# Autodesk Inventor assembly: Flywheel Gearbox
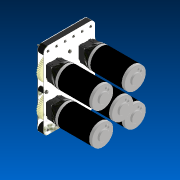
[picture p0: Inventor's stored thumbnail of the model, 180x180]
Saved by Autodesk Inventor 2022 (Build 260153000, 153)
## iProperties
Created: 2022-02-21
Part Number: Flywheel Gearbox
Document SubType Name: Assembly
Designer: omard
Mass: 7293.51 g
Surface Area: 6342.65 cm^2
Volume: 2548.68 cm^3
Density: 2.86168 g/cm^3
Author: omard
## Documents named in this file (21)
- C:\Users\score_nygvs6w\OneDrive - Auburn University\BasketBall Shooting Robot\Flywheel Gearbox.iam
- C:\Users\score_nygvs6w\OneDrive - Auburn University\BasketBall Shooting Robot\VEX Parts\CIM Motor (217-2000).ipt
- C:\Users\score_nygvs6w\OneDrive - Auburn University\BasketBall Shooting Robot\VEX Parts\VersaPlanetary v2 NoStage.iam
- C:\Users\score_nygvs6w\OneDrive - Auburn University\BasketBall Shooting Robot\VEX Parts\54T Aluminum Spur Gear (20 DP, 1_2 Hex Bore) (217-3573).ipt
- C:\Users\score_nygvs6w\OneDrive - Auburn University\BasketBall Shooting Robot\VEX Parts\54T Aluminum Spur Gear (20 DP, 1_2 Hex Bore, VersaKeys) (217-3221).ipt
- C:\Users\score_nygvs6w\OneDrive - Auburn University\BasketBall Shooting Robot\VEX Parts\Clamping Shaft Collar - 1_2 Hex ID (217-2737).ipt
- C:\Users\score_nygvs6w\OneDrive - Auburn University\BasketBall Shooting Robot\VEX Parts\60T x 18mm Wide VersaPulley Kit (HTD 5mm, VersaKeys) (217-3200).iam
- C:\Users\score_nygvs6w\OneDrive - Auburn University\BasketBall Shooting Robot\VEX Parts\1_2” Hex Bore Aluminum VersaHub (217-2592).ipt
- C:\Users\score_nygvs6w\OneDrive - Auburn University\BasketBall Shooting Robot\VEX Parts\1.125 Bearing Pilot Plastic VersaHub (1_4 Wide, w_ Plate Sprocket Mount) (217-3234).ipt
- C:\Users\score_nygvs6w\OneDrive - Auburn University\BasketBall Shooting Robot\Motor Bracket Outer Panel.ipt
- C:\Users\score_nygvs6w\OneDrive - Auburn University\BasketBall Shooting Robot\Motor Bracket Inner Panel.ipt
- C:\Users\score_nygvs6w\OneDrive - Auburn University\BasketBall Shooting Robot\VEX Parts\#8-32 x 0.625 Star Drive Screw (276-4993).ipt
- C:\Users\score_nygvs6w\OneDrive - Auburn University\BasketBall Shooting Robot\Motor Bracket Seperator.ipt
- C:\Users\score_nygvs6w\OneDrive - Auburn University\BasketBall Shooting Robot\VEX Parts\13.75mm (1_2 ThunderHex ID) x 1.125 OD x 0.313 WD (Flanged Bearing) (217-4006).ipt
- C:\Users\score_nygvs6w\OneDrive - Auburn University\BasketBall Shooting Robot\1_10 Spacer 1_2 Hex Custom.ipt
- C:\Users\score_nygvs6w\OneDrive - Auburn University\BasketBall Shooting Robot\VEX Parts\#8-32 x 1.250 Star Drive Screw (276-4997).ipt
- C:\Users\score_nygvs6w\OneDrive - Auburn University\BasketBall Shooting Robot\VEX Parts\#8-32 Nylock Nut (275-1027).ipt
- C:\Users\score_nygvs6w\OneDrive - Auburn University\BasketBall Shooting Robot\5_8 Spacer Screw Custom.ipt
- C:\Users\score_nygvs6w\OneDrive - Auburn University\BasketBall Shooting Robot\VEX Parts\#8-32 x 1.000 Star Drive Screw (276-4996).ipt
- C:\Users\score_nygvs6w\OneDrive - Auburn University\BasketBall Shooting Robot\VEX Parts\Falcon 500, Powered by Talon FX (217-6515).iam
- C:\Users\score_nygvs6w\OneDrive - Auburn University\BasketBall Shooting Robot\VEX Parts\VersaPlanetary v2 NoStage Encoder.iam
## Components (84 placed, 20 different names)
1. CIM Motor (217-2000):1 — Mate:5, Mate:6, Mate:18, Flush:10
2. CIM Motor (217-2000):2 — Flush:2, Mate:11, Mate:12, Mate:14, Mate:16, Mate:19, Mate:56
3. CIM Motor (217-2000):3 — Mate:7, Mate:8, Mate:15, Mate:18, Mate:19, Mate:54, Mate:55
4. CIM Motor (217-2000):4 — Flush:2, Mate:9, Mate:10, Mate:13, Mate:55, Flush:10, Flush:11
5. CIM Motor (217-2000):5 — Mate:54, Flush:11, Mate:56
6. VersaPlanetary v2 NoStage Encoder:1 [sub-assembly] — Angle:2, Mate:7, Mate:8, Mate:15, Mate:25, Angle:5, Mate:47, Angle:15, Mate:48, Mate:51, Angle:16, Mate:60, Mate:62, Angle:29, Mate:105, Mate:110, Angle:32, Mate:113, Mate:189, Mate:199
7. VersaPlanetary v2 NoStage:2 [sub-assembly] — Angle:3, Angle:4, Mate:11, Mate:12, Mate:14, Mate:23, Angle:7, Angle:10, Mate:59, Mate:99, Angle:30, Mate:106, Mate:112, Mate:187, Mate:193, Mate:200
8. VersaPlanetary v2 NoStage:3 [sub-assembly] — Mate:5, Angle:1, Angle:2, Angle:3, Mate:6, Mate:22, Angle:6, Mate:58, Mate:66, Mate:98, Angle:31, Mate:107, Mate:111, Mate:191, Mate:192, Mate:196, Mate:197, Flush:12
9. VersaPlanetary v2 NoStage:4 [sub-assembly] — Angle:4, Mate:9, Mate:10, Mate:13, Mate:24, Angle:8, Flush:8, Mate:57, Mate:97, Angle:27, Mate:103, Mate:108, Mate:190, Mate:195, Mate:198, Flush:12
10. VersaPlanetary v2 NoStage:5 [sub-assembly] — Flush:8, Angle:10, Mate:61, Mate:100, Angle:28, Mate:104, Mate:109, Mate:188, Mate:194, Mate:201, Mate:202
11. 54T Aluminum Spur Gear (20 DP, 1_2 Hex Bore) (217-3573):1 — Mate:22, Angle:6, Flush:6, Mate:102
12. 54T Aluminum Spur Gear (20 DP, 1_2 Hex Bore, VersaKeys) (217-3221):1 — Mate:25, Angle:5, Flush:4, Mate:49, Mate:50, Mate:52
13. 54T Aluminum Spur Gear (20 DP, 1_2 Hex Bore) (217-3573):2 — Mate:23, Angle:7, Flush:5, Flush:6
14. 54T Aluminum Spur Gear (20 DP, 1_2 Hex Bore) (217-3573):3 — Mate:24, Angle:8, Flush:4, Flush:5, Flush:7
15. 54T Aluminum Spur Gear (20 DP, 1_2 Hex Bore) (217-3573):4 — Flush:7
16. Clamping Shaft Collar - 1_2 Hex ID (217-2737):5 — Mate:51, Angle:16, Mate:52
17. 60T x 18mm Wide VersaPulley Kit (HTD 5mm, VersaKeys) (217-3200):1 [sub-assembly] — Mate:41, Mate:42, Mate:46, Mate:53, Mate:133, Mate:134, Mate:135, Mate:136, Mate:137, Mate:138, Angle:39, Angle:40, Angle:41, Angle:42, Angle:43, Angle:44
18. 1_2” Hex Bore Aluminum VersaHub (217-2592):1 — Mate:41, Mate:42, Mate:46, Mate:47, Angle:15, Mate:114, Mate:115, Mate:116, Mate:117, Mate:118, Mate:119, Mate:120, Mate:121, Mate:122, Mate:123, Mate:124, Mate:125, Mate:126
19. 1.125 Bearing Pilot Plastic VersaHub (1_4 Wide, w_ Plate Sprocket Mount) (217-3234):1 — Mate:48, Mate:49, Mate:50, Mate:53
20. Motor Bracket Outer Panel:1 — Mate:89, Mate:90, Mate:91, Mate:92, Mate:93, Mate:94, Mate:95, Mate:96, Mate:101, Mate:171, Mate:172, Mate:173, Mate:174, Mate:175, Mate:176, Mate:177, Mate:178, Angle:65, Angle:66, Angle:67, Angle:68
21. Motor Bracket Inner Panel:1 — Mate:57, Mate:58, Mate:59, Mate:60, Mate:61, Mate:62, Mate:63, Mate:64, Mate:65, Mate:67, Mate:68, Mate:69, Mate:70, Mate:71, Mate:72, Mate:73, Mate:74, Mate:75, Mate:76, Mate:77, Mate:78, Mate:79, Mate:80, Mate:81, Mate:82, Angle:17, Angle:18, Angle:19, Angle:20, Angle:21, Angle:22, Angle:23, Angle:24, Angle:25, Angle:26, Mate:83, Mate:84, Mate:85, Mate:86, Mate:87, Mate:88, Angle:33, Angle:34, Angle:35, Angle:36, Angle:37, Angle:38, Angle:45, Angle:46, Angle:47, Angle:48, Mate:139, Mate:140, Mate:141, Mate:142, Mate:143, Mate:144, Mate:145, Mate:146, Mate:147, Mate:148, Mate:149, Mate:150, Mate:151, Mate:152, Mate:153, Mate:154, Mate:155, Mate:156, Mate:157, Mate:158, Mate:159, Mate:160, Mate:161, Mate:162, Angle:49, Angle:50, Angle:51, Angle:52, Angle:53, Angle:54, Angle:55, Angle:56, Angle:57, Angle:58, Angle:59, Angle:60, Mate:163, Mate:164, Mate:165, Mate:166, Mate:167, Mate:168, Mate:169, Mate:170, Angle:61, Angle:62, Angle:63, Angle:64, Mate:183, Mate:184, Mate:185, Mate:186, Angle:69, Angle:70, Angle:71, Angle:72, Mate:202
22. #8-32 x 0.625 Star Drive Screw (276-4993):1 — Mate:65, Mate:81, Angle:26
23. #8-32 x 0.625 Star Drive Screw (276-4993):2 — Mate:66, Mate:82, Angle:25
24. #8-32 x 0.625 Star Drive Screw (276-4993):3 — Mate:63, Mate:80, Angle:24
25. #8-32 x 0.625 Star Drive Screw (276-4993):4 — Mate:64, Mate:79, Angle:23
26. #8-32 x 0.625 Star Drive Screw (276-4993):5 — Mate:72, Mate:73, Angle:22
27. #8-32 x 0.625 Star Drive Screw (276-4993):6 — Mate:71, Mate:74, Angle:21
28. #8-32 x 0.625 Star Drive Screw (276-4993):7 — Mate:68, Mate:76, Angle:20
29. #8-32 x 0.625 Star Drive Screw (276-4993):8 — Mate:67, Mate:75, Angle:19
30. #8-32 x 0.625 Star Drive Screw (276-4993):9 — Mate:70, Mate:78, Angle:18
31. #8-32 x 0.625 Star Drive Screw (276-4993):10 — Mate:69, Mate:77, Angle:17
32. Motor Bracket Seperator:1 — Mate:83, Mate:84, Mate:88
33. Motor Bracket Seperator:2 — Mate:85, Mate:86, Mate:87, Mate:101
34. 13.75mm (1_2 ThunderHex ID) x 1.125 OD x 0.313 WD (Flanged Bearing) (217-4006):1 — Mate:89, Mate:94, Mate:98, Mate:102, Angle:48
35. 13.75mm (1_2 ThunderHex ID) x 1.125 OD x 0.313 WD (Flanged Bearing) (217-4006):2 — Mate:90, Mate:95, Mate:97, Angle:47
36. 13.75mm (1_2 ThunderHex ID) x 1.125 OD x 0.313 WD (Flanged Bearing) (217-4006):3 — Mate:92, Mate:96, Mate:100, Angle:46
37. 13.75mm (1_2 ThunderHex ID) x 1.125 OD x 0.313 WD (Flanged Bearing) (217-4006):4 — Mate:91, Mate:93, Mate:99, Angle:45
38. 1_10 Spacer 1_2 Hex Custom:1 — Angle:27, Mate:104, Mate:109
39. 1_10 Spacer 1_2 Hex Custom:2 — Angle:30, Mate:106, Mate:112
40. 1_10 Spacer 1_2 Hex Custom:3 — Angle:31, Mate:107, Mate:111
41. 1_10 Spacer 1_2 Hex Custom:4 — Angle:29, Mate:105, Mate:110
42. 1_10 Spacer 1_2 Hex Custom:5 — Angle:28, Mate:103, Mate:108
43. 1_10 Spacer 1_2 Hex Custom:6 — Angle:32, Mate:113, Mate:114
44. #8-32 x 1.250 Star Drive Screw (276-4997):1 — Mate:120, Mate:124, Angle:38, Mate:127
45. #8-32 x 1.250 Star Drive Screw (276-4997):2 — Mate:116, Mate:123, Angle:37, Mate:128
46. #8-32 x 1.250 Star Drive Screw (276-4997):3 — Mate:118, Mate:125, Angle:36, Mate:130
47. #8-32 x 1.250 Star Drive Screw (276-4997):4 — Mate:115, Mate:121, Angle:35, Mate:131
48. #8-32 x 1.250 Star Drive Screw (276-4997):5 — Mate:117, Mate:122, Angle:34, Mate:132
49. #8-32 x 1.250 Star Drive Screw (276-4997):6 — Mate:119, Mate:126, Angle:33, Mate:129
50. #8-32 Nylock Nut (275-1027):1 — Mate:128, Mate:134, Angle:43
51. #8-32 Nylock Nut (275-1027):2 — Mate:129, Mate:136, Angle:42
52. #8-32 Nylock Nut (275-1027):3 — Mate:132, Mate:138, Angle:39
53. #8-32 Nylock Nut (275-1027):4 — Mate:131, Mate:133, Angle:40
54. #8-32 Nylock Nut (275-1027):5 — Mate:130, Mate:137, Angle:41
55. #8-32 Nylock Nut (275-1027):6 — Mate:127, Mate:135, Angle:44
56. #8-32 x 1.250 Star Drive Screw (276-4997):7 — Mate:144, Mate:162, Angle:60
57. #8-32 x 1.250 Star Drive Screw (276-4997):8 — Mate:143, Mate:161, Angle:58
58. #8-32 x 1.250 Star Drive Screw (276-4997):9 — Mate:141, Mate:159, Angle:59
59. #8-32 x 1.250 Star Drive Screw (276-4997):10 — Mate:140, Mate:158, Angle:57
60. #8-32 x 1.250 Star Drive Screw (276-4997):11 — Mate:142, Mate:160, Angle:56
61. #8-32 x 1.250 Star Drive Screw (276-4997):12 — Mate:139, Mate:157, Angle:55
62. #8-32 x 1.250 Star Drive Screw (276-4997):13 — Mate:145, Mate:151, Angle:54
63. #8-32 x 1.250 Star Drive Screw (276-4997):14 — Mate:146, Mate:152, Angle:53
64. #8-32 x 1.250 Star Drive Screw (276-4997):15 — Mate:147, Mate:153, Angle:52
65. #8-32 x 1.250 Star Drive Screw (276-4997):16 — Mate:148, Mate:154, Angle:51
66. #8-32 x 1.250 Star Drive Screw (276-4997):17 — Mate:149, Mate:155, Angle:50
67. #8-32 x 1.250 Star Drive Screw (276-4997):18 — Mate:150, Mate:156, Angle:49
68. 5_8 Spacer Screw Custom:1 — Mate:165, Mate:168, Angle:64
69. 5_8 Spacer Screw Custom:2 — Mate:166, Mate:167, Angle:63
70. 5_8 Spacer Screw Custom:3 — Mate:164, Mate:169, Angle:62
71. 5_8 Spacer Screw Custom:4 — Mate:163, Mate:170, Angle:61
72. #8-32 x 1.000 Star Drive Screw (276-4996):1 — Mate:171, Mate:172, Angle:65, Mate:181
73. #8-32 x 1.000 Star Drive Screw (276-4996):2 — Mate:173, Mate:174, Angle:66, Mate:179
74. #8-32 x 1.000 Star Drive Screw (276-4996):3 — Mate:177, Mate:178, Angle:68, Mate:182
75. #8-32 x 1.000 Star Drive Screw (276-4996):4 — Mate:175, Mate:176, Angle:67, Mate:180
76. #8-32 Nylock Nut (275-1027):7 — Mate:179, Mate:184, Angle:71
77. #8-32 Nylock Nut (275-1027):8 — Mate:180, Mate:183, Angle:72
78. #8-32 Nylock Nut (275-1027):9 — Mate:181, Mate:185, Angle:70
79. #8-32 Nylock Nut (275-1027):10 — Mate:182, Mate:186, Angle:69
80. Falcon 500, Powered by Talon FX (217-6515):1 [sub-assembly] — Mate:187, Mate:193, Mate:200
81. Falcon 500, Powered by Talon FX (217-6515):2 [sub-assembly] — Mate:189, Mate:199
82. Falcon 500, Powered by Talon FX (217-6515):3 [sub-assembly] — Mate:190, Mate:195, Mate:198
83. Falcon 500, Powered by Talon FX (217-6515):4 [sub-assembly] — Mate:191, Mate:192, Mate:196, Mate:197
84. Falcon 500, Powered by Talon FX (217-6515):5 [sub-assembly] — Mate:188, Mate:194, Mate:201
## Relationships (258: Mate 181, Angle 68, Flush 9)
- Flush:2: CIM Motor (217-2000):2 ↔ CIM Motor (217-2000):4
- Mate:5: CIM Motor (217-2000):1 ↔ VersaPlanetary v2 NoStage:3
- Angle:1 (0 deg): VersaPlanetary v2 NoStage:3
- Angle:2 (0 deg): VersaPlanetary v2 NoStage Encoder:1 ↔ VersaPlanetary v2 NoStage:3
- Angle:3 (0 deg): VersaPlanetary v2 NoStage:2 ↔ VersaPlanetary v2 NoStage:3
- Angle:4 (0 deg): VersaPlanetary v2 NoStage:2 ↔ VersaPlanetary v2 NoStage:4
- Mate:6: CIM Motor (217-2000):1 ↔ VersaPlanetary v2 NoStage:3
- Mate:7: CIM Motor (217-2000):3 ↔ VersaPlanetary v2 NoStage Encoder:1
- Mate:8: CIM Motor (217-2000):3 ↔ VersaPlanetary v2 NoStage Encoder:1
- Mate:9: CIM Motor (217-2000):4 ↔ VersaPlanetary v2 NoStage:4
- Mate:10: CIM Motor (217-2000):4 ↔ VersaPlanetary v2 NoStage:4
- Mate:11: CIM Motor (217-2000):2 ↔ VersaPlanetary v2 NoStage:2
- Mate:12: CIM Motor (217-2000):2 ↔ VersaPlanetary v2 NoStage:2
- Mate:13: CIM Motor (217-2000):4 ↔ VersaPlanetary v2 NoStage:4
- Mate:14: CIM Motor (217-2000):2 ↔ VersaPlanetary v2 NoStage:2
- Mate:15: CIM Motor (217-2000):3 ↔ VersaPlanetary v2 NoStage Encoder:1
- Mate:16: CIM Motor (217-2000):2
- Mate:18 (68.58 mm): CIM Motor (217-2000):1 ↔ CIM Motor (217-2000):3
- Mate:19 (68.58 mm): CIM Motor (217-2000):2 ↔ CIM Motor (217-2000):3
- Mate:22: VersaPlanetary v2 NoStage:3 ↔ 54T Aluminum Spur Gear (20 DP, 1_2 Hex Bore) (217-3573):1
- Mate:23: VersaPlanetary v2 NoStage:2 ↔ 54T Aluminum Spur Gear (20 DP, 1_2 Hex Bore) (217-3573):2
- Mate:24: VersaPlanetary v2 NoStage:4 ↔ 54T Aluminum Spur Gear (20 DP, 1_2 Hex Bore) (217-3573):3
- Mate:25: VersaPlanetary v2 NoStage Encoder:1 ↔ 54T Aluminum Spur Gear (20 DP, 1_2 Hex Bore, VersaKeys) (217-3221):1
- Angle:5 (0 deg): VersaPlanetary v2 NoStage Encoder:1 ↔ 54T Aluminum Spur Gear (20 DP, 1_2 Hex Bore, VersaKeys) (217-3221):1
- Angle:6 (0 deg): VersaPlanetary v2 NoStage:3 ↔ 54T Aluminum Spur Gear (20 DP, 1_2 Hex Bore) (217-3573):1
- Angle:7 (0 deg): VersaPlanetary v2 NoStage:2 ↔ 54T Aluminum Spur Gear (20 DP, 1_2 Hex Bore) (217-3573):2
- Angle:8 (0 deg): VersaPlanetary v2 NoStage:4 ↔ 54T Aluminum Spur Gear (20 DP, 1_2 Hex Bore) (217-3573):3
- Flush:4: 54T Aluminum Spur Gear (20 DP, 1_2 Hex Bore, VersaKeys) (217-3221):1 ↔ 54T Aluminum Spur Gear (20 DP, 1_2 Hex Bore) (217-3573):3
- Flush:5: 54T Aluminum Spur Gear (20 DP, 1_2 Hex Bore) (217-3573):2 ↔ 54T Aluminum Spur Gear (20 DP, 1_2 Hex Bore) (217-3573):3
- Flush:6: 54T Aluminum Spur Gear (20 DP, 1_2 Hex Bore) (217-3573):1 ↔ 54T Aluminum Spur Gear (20 DP, 1_2 Hex Bore) (217-3573):2
- [Mate]: CIM Motor (217-2000):5 ↔ VersaPlanetary v2 NoStage:5
- [Mate]: CIM Motor (217-2000):5 ↔ VersaPlanetary v2 NoStage:5
- [Mate]: CIM Motor (217-2000):5 ↔ VersaPlanetary v2 NoStage:5
- [Mate]: VersaPlanetary v2 NoStage:5 ↔ 54T Aluminum Spur Gear (20 DP, 1_2 Hex Bore) (217-3573):4
- [Angle] (0 deg): VersaPlanetary v2 NoStage:5 ↔ 54T Aluminum Spur Gear (20 DP, 1_2 Hex Bore) (217-3573):4
- Flush:7: 54T Aluminum Spur Gear (20 DP, 1_2 Hex Bore) (217-3573):3 ↔ 54T Aluminum Spur Gear (20 DP, 1_2 Hex Bore) (217-3573):4
- Flush:8: VersaPlanetary v2 NoStage:4 ↔ VersaPlanetary v2 NoStage:5
- Angle:10 (0 deg): VersaPlanetary v2 NoStage:2 ↔ VersaPlanetary v2 NoStage:5
- Mate:41: 60T x 18mm Wide VersaPulley Kit (HTD 5mm, VersaKeys) (217-3200):1 ↔ 1_2” Hex Bore Aluminum VersaHub (217-2592):1
- Mate:42: 60T x 18mm Wide VersaPulley Kit (HTD 5mm, VersaKeys) (217-3200):1 ↔ 1_2” Hex Bore Aluminum VersaHub (217-2592):1
- Mate:46: 60T x 18mm Wide VersaPulley Kit (HTD 5mm, VersaKeys) (217-3200):1 ↔ 1_2” Hex Bore Aluminum VersaHub (217-2592):1
- Mate:47: VersaPlanetary v2 NoStage Encoder:1 ↔ 1_2” Hex Bore Aluminum VersaHub (217-2592):1
- Angle:15 (0 deg): VersaPlanetary v2 NoStage Encoder:1 ↔ 1_2” Hex Bore Aluminum VersaHub (217-2592):1
- Mate:48: VersaPlanetary v2 NoStage Encoder:1 ↔ 1.125 Bearing Pilot Plastic VersaHub (1_4 Wide, w_ Plate Sprocket Mount) (217-3234):1
- Mate:49: 54T Aluminum Spur Gear (20 DP, 1_2 Hex Bore, VersaKeys) (217-3221):1 ↔ 1.125 Bearing Pilot Plastic VersaHub (1_4 Wide, w_ Plate Sprocket Mount) (217-3234):1
- Mate:50: 54T Aluminum Spur Gear (20 DP, 1_2 Hex Bore, VersaKeys) (217-3221):1 ↔ 1.125 Bearing Pilot Plastic VersaHub (1_4 Wide, w_ Plate Sprocket Mount) (217-3234):1
- Mate:51: VersaPlanetary v2 NoStage Encoder:1 ↔ Clamping Shaft Collar - 1_2 Hex ID (217-2737):5
- Angle:16 (0 deg): VersaPlanetary v2 NoStage Encoder:1 ↔ Clamping Shaft Collar - 1_2 Hex ID (217-2737):5
- Mate:52: 54T Aluminum Spur Gear (20 DP, 1_2 Hex Bore, VersaKeys) (217-3221):1 ↔ Clamping Shaft Collar - 1_2 Hex ID (217-2737):5
- Mate:53: 60T x 18mm Wide VersaPulley Kit (HTD 5mm, VersaKeys) (217-3200):1 ↔ 1.125 Bearing Pilot Plastic VersaHub (1_4 Wide, w_ Plate Sprocket Mount) (217-3234):1
- Mate:54 (68.58 mm): CIM Motor (217-2000):3 ↔ CIM Motor (217-2000):5
- Mate:55 (68.58 mm): CIM Motor (217-2000):3 ↔ CIM Motor (217-2000):4
- Flush:10: CIM Motor (217-2000):1 ↔ CIM Motor (217-2000):4
- Flush:11: CIM Motor (217-2000):4 ↔ CIM Motor (217-2000):5
- Mate:56 (96.9868 mm): CIM Motor (217-2000):2 ↔ CIM Motor (217-2000):5
- Mate:57: VersaPlanetary v2 NoStage:4 ↔ Motor Bracket Inner Panel:1
- Mate:58: VersaPlanetary v2 NoStage:3 ↔ Motor Bracket Inner Panel:1
- Mate:59: VersaPlanetary v2 NoStage:2 ↔ Motor Bracket Inner Panel:1
- Mate:60: VersaPlanetary v2 NoStage Encoder:1 ↔ Motor Bracket Inner Panel:1
- Mate:61: VersaPlanetary v2 NoStage:5 ↔ Motor Bracket Inner Panel:1
- Mate:62: VersaPlanetary v2 NoStage Encoder:1 ↔ Motor Bracket Inner Panel:1
- Mate:63: Motor Bracket Inner Panel:1 ↔ #8-32 x 0.625 Star Drive Screw (276-4993):3
- Mate:64: Motor Bracket Inner Panel:1 ↔ #8-32 x 0.625 Star Drive Screw (276-4993):4
- Mate:65: Motor Bracket Inner Panel:1 ↔ #8-32 x 0.625 Star Drive Screw (276-4993):1
- Mate:66: VersaPlanetary v2 NoStage:3 ↔ #8-32 x 0.625 Star Drive Screw (276-4993):2
- Mate:67: Motor Bracket Inner Panel:1 ↔ #8-32 x 0.625 Star Drive Screw (276-4993):8
- Mate:68: Motor Bracket Inner Panel:1 ↔ #8-32 x 0.625 Star Drive Screw (276-4993):7
- Mate:69: Motor Bracket Inner Panel:1 ↔ #8-32 x 0.625 Star Drive Screw (276-4993):10
- Mate:70: Motor Bracket Inner Panel:1 ↔ #8-32 x 0.625 Star Drive Screw (276-4993):9
- Mate:71: Motor Bracket Inner Panel:1 ↔ #8-32 x 0.625 Star Drive Screw (276-4993):6
- Mate:72: Motor Bracket Inner Panel:1 ↔ #8-32 x 0.625 Star Drive Screw (276-4993):5
- Mate:73: Motor Bracket Inner Panel:1 ↔ #8-32 x 0.625 Star Drive Screw (276-4993):5
- Mate:74: Motor Bracket Inner Panel:1 ↔ #8-32 x 0.625 Star Drive Screw (276-4993):6
- Mate:75: Motor Bracket Inner Panel:1 ↔ #8-32 x 0.625 Star Drive Screw (276-4993):8
- Mate:76: Motor Bracket Inner Panel:1 ↔ #8-32 x 0.625 Star Drive Screw (276-4993):7
- Mate:77: Motor Bracket Inner Panel:1 ↔ #8-32 x 0.625 Star Drive Screw (276-4993):10
- Mate:78: Motor Bracket Inner Panel:1 ↔ #8-32 x 0.625 Star Drive Screw (276-4993):9
- Mate:79: Motor Bracket Inner Panel:1 ↔ #8-32 x 0.625 Star Drive Screw (276-4993):4
- Mate:80: Motor Bracket Inner Panel:1 ↔ #8-32 x 0.625 Star Drive Screw (276-4993):3
- Mate:81: Motor Bracket Inner Panel:1 ↔ #8-32 x 0.625 Star Drive Screw (276-4993):1
- Mate:82: Motor Bracket Inner Panel:1 ↔ #8-32 x 0.625 Star Drive Screw (276-4993):2
- Angle:17 (0 deg): Motor Bracket Inner Panel:1 ↔ #8-32 x 0.625 Star Drive Screw (276-4993):10
- Angle:18 (0 deg): Motor Bracket Inner Panel:1 ↔ #8-32 x 0.625 Star Drive Screw (276-4993):9
- Angle:19 (0 deg): Motor Bracket Inner Panel:1 ↔ #8-32 x 0.625 Star Drive Screw (276-4993):8
- Angle:20 (0 deg): Motor Bracket Inner Panel:1 ↔ #8-32 x 0.625 Star Drive Screw (276-4993):7
- Angle:21 (0 deg): Motor Bracket Inner Panel:1 ↔ #8-32 x 0.625 Star Drive Screw (276-4993):6
- Angle:22 (0 deg): Motor Bracket Inner Panel:1 ↔ #8-32 x 0.625 Star Drive Screw (276-4993):5
- Angle:23 (0 deg): Motor Bracket Inner Panel:1 ↔ #8-32 x 0.625 Star Drive Screw (276-4993):4
- Angle:24 (0 deg): Motor Bracket Inner Panel:1 ↔ #8-32 x 0.625 Star Drive Screw (276-4993):3
- Angle:25 (0 deg): Motor Bracket Inner Panel:1 ↔ #8-32 x 0.625 Star Drive Screw (276-4993):2
- Angle:26 (0 deg): Motor Bracket Inner Panel:1 ↔ #8-32 x 0.625 Star Drive Screw (276-4993):1
- Mate:83: Motor Bracket Inner Panel:1 ↔ Motor Bracket Seperator:1
- Mate:84: Motor Bracket Inner Panel:1 ↔ Motor Bracket Seperator:1
- Mate:85: Motor Bracket Inner Panel:1 ↔ Motor Bracket Seperator:2
- Mate:86: Motor Bracket Inner Panel:1 ↔ Motor Bracket Seperator:2
- Mate:87: Motor Bracket Inner Panel:1 ↔ Motor Bracket Seperator:2
- Mate:88: Motor Bracket Inner Panel:1 ↔ Motor Bracket Seperator:1
- Mate:89: Motor Bracket Outer Panel:1 ↔ 13.75mm (1_2 ThunderHex ID) x 1.125 OD x 0.313 WD (Flanged Bearing) (217-4006):1
- Mate:90: Motor Bracket Outer Panel:1 ↔ 13.75mm (1_2 ThunderHex ID) x 1.125 OD x 0.313 WD (Flanged Bearing) (217-4006):2
- Mate:91: Motor Bracket Outer Panel:1 ↔ 13.75mm (1_2 ThunderHex ID) x 1.125 OD x 0.313 WD (Flanged Bearing) (217-4006):4
- Mate:92: Motor Bracket Outer Panel:1 ↔ 13.75mm (1_2 ThunderHex ID) x 1.125 OD x 0.313 WD (Flanged Bearing) (217-4006):3
- Mate:93: Motor Bracket Outer Panel:1 ↔ 13.75mm (1_2 ThunderHex ID) x 1.125 OD x 0.313 WD (Flanged Bearing) (217-4006):4
- Mate:94: Motor Bracket Outer Panel:1 ↔ 13.75mm (1_2 ThunderHex ID) x 1.125 OD x 0.313 WD (Flanged Bearing) (217-4006):1
- Mate:95: Motor Bracket Outer Panel:1 ↔ 13.75mm (1_2 ThunderHex ID) x 1.125 OD x 0.313 WD (Flanged Bearing) (217-4006):2
- Mate:96: Motor Bracket Outer Panel:1 ↔ 13.75mm (1_2 ThunderHex ID) x 1.125 OD x 0.313 WD (Flanged Bearing) (217-4006):3
- Mate:97: VersaPlanetary v2 NoStage:4 ↔ 13.75mm (1_2 ThunderHex ID) x 1.125 OD x 0.313 WD (Flanged Bearing) (217-4006):2
- Mate:98: VersaPlanetary v2 NoStage:3 ↔ 13.75mm (1_2 ThunderHex ID) x 1.125 OD x 0.313 WD (Flanged Bearing) (217-4006):1
- Mate:99: VersaPlanetary v2 NoStage:2 ↔ 13.75mm (1_2 ThunderHex ID) x 1.125 OD x 0.313 WD (Flanged Bearing) (217-4006):4
- Mate:100: VersaPlanetary v2 NoStage:5 ↔ 13.75mm (1_2 ThunderHex ID) x 1.125 OD x 0.313 WD (Flanged Bearing) (217-4006):3
- Mate:101: Motor Bracket Outer Panel:1 ↔ Motor Bracket Seperator:2
- Mate:102: 54T Aluminum Spur Gear (20 DP, 1_2 Hex Bore) (217-3573):1 ↔ 13.75mm (1_2 ThunderHex ID) x 1.125 OD x 0.313 WD (Flanged Bearing) (217-4006):1
- Angle:27 (0 deg): VersaPlanetary v2 NoStage:4 ↔ 1_10 Spacer 1_2 Hex Custom:1
- Angle:28 (0 deg): VersaPlanetary v2 NoStage:5 ↔ 1_10 Spacer 1_2 Hex Custom:5
- Angle:29 (0 deg): VersaPlanetary v2 NoStage Encoder:1 ↔ 1_10 Spacer 1_2 Hex Custom:4
- Angle:30 (0 deg): VersaPlanetary v2 NoStage:2 ↔ 1_10 Spacer 1_2 Hex Custom:2
- Angle:31 (0 deg): VersaPlanetary v2 NoStage:3 ↔ 1_10 Spacer 1_2 Hex Custom:3
- Mate:103: VersaPlanetary v2 NoStage:4 ↔ 1_10 Spacer 1_2 Hex Custom:5
- Mate:104: VersaPlanetary v2 NoStage:5 ↔ 1_10 Spacer 1_2 Hex Custom:1
- Mate:105: VersaPlanetary v2 NoStage Encoder:1 ↔ 1_10 Spacer 1_2 Hex Custom:4
- Mate:106: VersaPlanetary v2 NoStage:2 ↔ 1_10 Spacer 1_2 Hex Custom:2
- Mate:107: VersaPlanetary v2 NoStage:3 ↔ 1_10 Spacer 1_2 Hex Custom:3
- Mate:108: VersaPlanetary v2 NoStage:4 ↔ 1_10 Spacer 1_2 Hex Custom:5
- Mate:109: VersaPlanetary v2 NoStage:5 ↔ 1_10 Spacer 1_2 Hex Custom:1
- Mate:110: VersaPlanetary v2 NoStage Encoder:1 ↔ 1_10 Spacer 1_2 Hex Custom:4
- Mate:111: VersaPlanetary v2 NoStage:3 ↔ 1_10 Spacer 1_2 Hex Custom:3
- Mate:112: VersaPlanetary v2 NoStage:2 ↔ 1_10 Spacer 1_2 Hex Custom:2
- Angle:32 (0 deg): VersaPlanetary v2 NoStage Encoder:1 ↔ 1_10 Spacer 1_2 Hex Custom:6
- Mate:113: VersaPlanetary v2 NoStage Encoder:1 ↔ 1_10 Spacer 1_2 Hex Custom:6
- Mate:114: 1_2” Hex Bore Aluminum VersaHub (217-2592):1 ↔ 1_10 Spacer 1_2 Hex Custom:6
- Mate:115: 1_2” Hex Bore Aluminum VersaHub (217-2592):1 ↔ #8-32 x 1.250 Star Drive Screw (276-4997):4
- Mate:116: 1_2” Hex Bore Aluminum VersaHub (217-2592):1 ↔ #8-32 x 1.250 Star Drive Screw (276-4997):2
- Mate:117: 1_2” Hex Bore Aluminum VersaHub (217-2592):1 ↔ #8-32 x 1.250 Star Drive Screw (276-4997):5
- Mate:118: 1_2” Hex Bore Aluminum VersaHub (217-2592):1 ↔ #8-32 x 1.250 Star Drive Screw (276-4997):3
- Mate:119: 1_2” Hex Bore Aluminum VersaHub (217-2592):1 ↔ #8-32 x 1.250 Star Drive Screw (276-4997):6
- Mate:120: 1_2” Hex Bore Aluminum VersaHub (217-2592):1 ↔ #8-32 x 1.250 Star Drive Screw (276-4997):1
- Mate:121: 1_2” Hex Bore Aluminum VersaHub (217-2592):1 ↔ #8-32 x 1.250 Star Drive Screw (276-4997):4
- Mate:122: 1_2” Hex Bore Aluminum VersaHub (217-2592):1 ↔ #8-32 x 1.250 Star Drive Screw (276-4997):5
- Mate:123: 1_2” Hex Bore Aluminum VersaHub (217-2592):1 ↔ #8-32 x 1.250 Star Drive Screw (276-4997):2
- Mate:124: 1_2” Hex Bore Aluminum VersaHub (217-2592):1 ↔ #8-32 x 1.250 Star Drive Screw (276-4997):1
- Mate:125: 1_2” Hex Bore Aluminum VersaHub (217-2592):1 ↔ #8-32 x 1.250 Star Drive Screw (276-4997):3
- Mate:126: 1_2” Hex Bore Aluminum VersaHub (217-2592):1 ↔ #8-32 x 1.250 Star Drive Screw (276-4997):6
- Angle:33 (0 deg): Motor Bracket Inner Panel:1 ↔ #8-32 x 1.250 Star Drive Screw (276-4997):6
- Angle:34 (0 deg): Motor Bracket Inner Panel:1 ↔ #8-32 x 1.250 Star Drive Screw (276-4997):5
- Angle:35 (0 deg): Motor Bracket Inner Panel:1 ↔ #8-32 x 1.250 Star Drive Screw (276-4997):4
- Angle:36 (0 deg): Motor Bracket Inner Panel:1 ↔ #8-32 x 1.250 Star Drive Screw (276-4997):3
- Angle:37 (0 deg): Motor Bracket Inner Panel:1 ↔ #8-32 x 1.250 Star Drive Screw (276-4997):2
- Angle:38 (0 deg): Motor Bracket Inner Panel:1 ↔ #8-32 x 1.250 Star Drive Screw (276-4997):1
- Mate:127: #8-32 x 1.250 Star Drive Screw (276-4997):1 ↔ #8-32 Nylock Nut (275-1027):6
- Mate:128: #8-32 x 1.250 Star Drive Screw (276-4997):2 ↔ #8-32 Nylock Nut (275-1027):1
- Mate:129: #8-32 x 1.250 Star Drive Screw (276-4997):6 ↔ #8-32 Nylock Nut (275-1027):2
- Mate:130: #8-32 x 1.250 Star Drive Screw (276-4997):3 ↔ #8-32 Nylock Nut (275-1027):5
- Mate:131: #8-32 x 1.250 Star Drive Screw (276-4997):4 ↔ #8-32 Nylock Nut (275-1027):4
- Mate:132: #8-32 x 1.250 Star Drive Screw (276-4997):5 ↔ #8-32 Nylock Nut (275-1027):3
- Mate:133: 60T x 18mm Wide VersaPulley Kit (HTD 5mm, VersaKeys) (217-3200):1 ↔ #8-32 Nylock Nut (275-1027):4
- Mate:134: 60T x 18mm Wide VersaPulley Kit (HTD 5mm, VersaKeys) (217-3200):1 ↔ #8-32 Nylock Nut (275-1027):1
- Mate:135: 60T x 18mm Wide VersaPulley Kit (HTD 5mm, VersaKeys) (217-3200):1 ↔ #8-32 Nylock Nut (275-1027):6
- Mate:136: 60T x 18mm Wide VersaPulley Kit (HTD 5mm, VersaKeys) (217-3200):1 ↔ #8-32 Nylock Nut (275-1027):2
- Mate:137: 60T x 18mm Wide VersaPulley Kit (HTD 5mm, VersaKeys) (217-3200):1 ↔ #8-32 Nylock Nut (275-1027):5
- Mate:138: 60T x 18mm Wide VersaPulley Kit (HTD 5mm, VersaKeys) (217-3200):1 ↔ #8-32 Nylock Nut (275-1027):3
- Angle:39 (0 deg): 60T x 18mm Wide VersaPulley Kit (HTD 5mm, VersaKeys) (217-3200):1 ↔ #8-32 Nylock Nut (275-1027):3
- Angle:40 (0 deg): 60T x 18mm Wide VersaPulley Kit (HTD 5mm, VersaKeys) (217-3200):1 ↔ #8-32 Nylock Nut (275-1027):4
- Angle:41 (0 deg): 60T x 18mm Wide VersaPulley Kit (HTD 5mm, VersaKeys) (217-3200):1 ↔ #8-32 Nylock Nut (275-1027):5
- Angle:42 (0 deg): 60T x 18mm Wide VersaPulley Kit (HTD 5mm, VersaKeys) (217-3200):1 ↔ #8-32 Nylock Nut (275-1027):2
- Angle:43 (0 deg): 60T x 18mm Wide VersaPulley Kit (HTD 5mm, VersaKeys) (217-3200):1 ↔ #8-32 Nylock Nut (275-1027):1
- Angle:44 (0 deg): 60T x 18mm Wide VersaPulley Kit (HTD 5mm, VersaKeys) (217-3200):1 ↔ #8-32 Nylock Nut (275-1027):6
- Angle:45 (0 deg): Motor Bracket Inner Panel:1 ↔ 13.75mm (1_2 ThunderHex ID) x 1.125 OD x 0.313 WD (Flanged Bearing) (217-4006):4
- Angle:46 (0 deg): Motor Bracket Inner Panel:1 ↔ 13.75mm (1_2 ThunderHex ID) x 1.125 OD x 0.313 WD (Flanged Bearing) (217-4006):3
- Angle:47 (0 deg): Motor Bracket Inner Panel:1 ↔ 13.75mm (1_2 ThunderHex ID) x 1.125 OD x 0.313 WD (Flanged Bearing) (217-4006):2
- Angle:48 (0 deg): Motor Bracket Inner Panel:1 ↔ 13.75mm (1_2 ThunderHex ID) x 1.125 OD x 0.313 WD (Flanged Bearing) (217-4006):1
- Mate:139: Motor Bracket Inner Panel:1 ↔ #8-32 x 1.250 Star Drive Screw (276-4997):12
- Mate:140: Motor Bracket Inner Panel:1 ↔ #8-32 x 1.250 Star Drive Screw (276-4997):10
- Mate:141: Motor Bracket Inner Panel:1 ↔ #8-32 x 1.250 Star Drive Screw (276-4997):9
- Mate:142: Motor Bracket Inner Panel:1 ↔ #8-32 x 1.250 Star Drive Screw (276-4997):11
- Mate:143: Motor Bracket Inner Panel:1 ↔ #8-32 x 1.250 Star Drive Screw (276-4997):8
- Mate:144: Motor Bracket Inner Panel:1 ↔ #8-32 x 1.250 Star Drive Screw (276-4997):7
- Mate:145: Motor Bracket Inner Panel:1 ↔ #8-32 x 1.250 Star Drive Screw (276-4997):13
- Mate:146: Motor Bracket Inner Panel:1 ↔ #8-32 x 1.250 Star Drive Screw (276-4997):14
- Mate:147: Motor Bracket Inner Panel:1 ↔ #8-32 x 1.250 Star Drive Screw (276-4997):15
- Mate:148: Motor Bracket Inner Panel:1 ↔ #8-32 x 1.250 Star Drive Screw (276-4997):16
- Mate:149: Motor Bracket Inner Panel:1 ↔ #8-32 x 1.250 Star Drive Screw (276-4997):17
- Mate:150: Motor Bracket Inner Panel:1 ↔ #8-32 x 1.250 Star Drive Screw (276-4997):18
- Mate:151: Motor Bracket Inner Panel:1 ↔ #8-32 x 1.250 Star Drive Screw (276-4997):13
- Mate:152: Motor Bracket Inner Panel:1 ↔ #8-32 x 1.250 Star Drive Screw (276-4997):14
- Mate:153: Motor Bracket Inner Panel:1 ↔ #8-32 x 1.250 Star Drive Screw (276-4997):15
- Mate:154: Motor Bracket Inner Panel:1 ↔ #8-32 x 1.250 Star Drive Screw (276-4997):16
- Mate:155: Motor Bracket Inner Panel:1 ↔ #8-32 x 1.250 Star Drive Screw (276-4997):17
- Mate:156: Motor Bracket Inner Panel:1 ↔ #8-32 x 1.250 Star Drive Screw (276-4997):18
- Mate:157: Motor Bracket Inner Panel:1 ↔ #8-32 x 1.250 Star Drive Screw (276-4997):12
- Mate:158: Motor Bracket Inner Panel:1 ↔ #8-32 x 1.250 Star Drive Screw (276-4997):10
- Mate:159: Motor Bracket Inner Panel:1 ↔ #8-32 x 1.250 Star Drive Screw (276-4997):9
- Mate:160: Motor Bracket Inner Panel:1 ↔ #8-32 x 1.250 Star Drive Screw (276-4997):11
- Mate:161: Motor Bracket Inner Panel:1 ↔ #8-32 x 1.250 Star Drive Screw (276-4997):8
- Mate:162: Motor Bracket Inner Panel:1 ↔ #8-32 x 1.250 Star Drive Screw (276-4997):7
- Angle:49 (0 deg): Motor Bracket Inner Panel:1 ↔ #8-32 x 1.250 Star Drive Screw (276-4997):18
- Angle:50 (0 deg): Motor Bracket Inner Panel:1 ↔ #8-32 x 1.250 Star Drive Screw (276-4997):17
- Angle:51 (0 deg): Motor Bracket Inner Panel:1 ↔ #8-32 x 1.250 Star Drive Screw (276-4997):16
- Angle:52 (0 deg): Motor Bracket Inner Panel:1 ↔ #8-32 x 1.250 Star Drive Screw (276-4997):15
- Angle:53 (0 deg): Motor Bracket Inner Panel:1 ↔ #8-32 x 1.250 Star Drive Screw (276-4997):14
- Angle:54 (0 deg): Motor Bracket Inner Panel:1 ↔ #8-32 x 1.250 Star Drive Screw (276-4997):13
- Angle:55 (0 deg): Motor Bracket Inner Panel:1 ↔ #8-32 x 1.250 Star Drive Screw (276-4997):12
- Angle:56 (0 deg): Motor Bracket Inner Panel:1 ↔ #8-32 x 1.250 Star Drive Screw (276-4997):11
- Angle:57 (0 deg): Motor Bracket Inner Panel:1 ↔ #8-32 x 1.250 Star Drive Screw (276-4997):10
- Angle:58 (0 deg): Motor Bracket Inner Panel:1 ↔ #8-32 x 1.250 Star Drive Screw (276-4997):8
- Angle:59 (0 deg): Motor Bracket Inner Panel:1 ↔ #8-32 x 1.250 Star Drive Screw (276-4997):9
- Angle:60 (0 deg): Motor Bracket Inner Panel:1 ↔ #8-32 x 1.250 Star Drive Screw (276-4997):7
- Mate:163: Motor Bracket Inner Panel:1 ↔ 5_8 Spacer Screw Custom:4
- Mate:164: Motor Bracket Inner Panel:1 ↔ 5_8 Spacer Screw Custom:3
- Mate:165: Motor Bracket Inner Panel:1 ↔ 5_8 Spacer Screw Custom:1
- Mate:166: Motor Bracket Inner Panel:1 ↔ 5_8 Spacer Screw Custom:2
- Mate:167: Motor Bracket Inner Panel:1 ↔ 5_8 Spacer Screw Custom:2
- Mate:168: Motor Bracket Inner Panel:1 ↔ 5_8 Spacer Screw Custom:1
- Mate:169: Motor Bracket Inner Panel:1 ↔ 5_8 Spacer Screw Custom:3
- Mate:170: Motor Bracket Inner Panel:1 ↔ 5_8 Spacer Screw Custom:4
- Angle:61 (0 deg): Motor Bracket Inner Panel:1 ↔ 5_8 Spacer Screw Custom:4
- Angle:62 (0 deg): Motor Bracket Inner Panel:1 ↔ 5_8 Spacer Screw Custom:3
- Angle:63 (0 deg): Motor Bracket Inner Panel:1 ↔ 5_8 Spacer Screw Custom:2
- Angle:64 (0 deg): Motor Bracket Inner Panel:1 ↔ 5_8 Spacer Screw Custom:1
- Mate:171: Motor Bracket Outer Panel:1 ↔ #8-32 x 1.000 Star Drive Screw (276-4996):1
- Mate:172: Motor Bracket Outer Panel:1 ↔ #8-32 x 1.000 Star Drive Screw (276-4996):1
- Mate:173: Motor Bracket Outer Panel:1 ↔ #8-32 x 1.000 Star Drive Screw (276-4996):2
- Mate:174: Motor Bracket Outer Panel:1 ↔ #8-32 x 1.000 Star Drive Screw (276-4996):2
- Mate:175: Motor Bracket Outer Panel:1 ↔ #8-32 x 1.000 Star Drive Screw (276-4996):4
- Mate:176: Motor Bracket Outer Panel:1 ↔ #8-32 x 1.000 Star Drive Screw (276-4996):4
- Mate:177: Motor Bracket Outer Panel:1 ↔ #8-32 x 1.000 Star Drive Screw (276-4996):3
- Mate:178: Motor Bracket Outer Panel:1 ↔ #8-32 x 1.000 Star Drive Screw (276-4996):3
- Angle:65 (0 deg): Motor Bracket Outer Panel:1 ↔ #8-32 x 1.000 Star Drive Screw (276-4996):1
- Angle:66 (0 deg): Motor Bracket Outer Panel:1 ↔ #8-32 x 1.000 Star Drive Screw (276-4996):2
- Angle:67 (0 deg): Motor Bracket Outer Panel:1 ↔ #8-32 x 1.000 Star Drive Screw (276-4996):4
- Angle:68 (0 deg): Motor Bracket Outer Panel:1 ↔ #8-32 x 1.000 Star Drive Screw (276-4996):3
- Mate:179: #8-32 x 1.000 Star Drive Screw (276-4996):2 ↔ #8-32 Nylock Nut (275-1027):7
- Mate:180: #8-32 x 1.000 Star Drive Screw (276-4996):4 ↔ #8-32 Nylock Nut (275-1027):8
- Mate:181: #8-32 x 1.000 Star Drive Screw (276-4996):1 ↔ #8-32 Nylock Nut (275-1027):9
- Mate:182: #8-32 x 1.000 Star Drive Screw (276-4996):3 ↔ #8-32 Nylock Nut (275-1027):10
- Mate:183: Motor Bracket Inner Panel:1 ↔ #8-32 Nylock Nut (275-1027):8
- Mate:184: Motor Bracket Inner Panel:1 ↔ #8-32 Nylock Nut (275-1027):7
- Mate:185: Motor Bracket Inner Panel:1 ↔ #8-32 Nylock Nut (275-1027):9
- Mate:186: Motor Bracket Inner Panel:1 ↔ #8-32 Nylock Nut (275-1027):10
- Angle:69 (0 deg): Motor Bracket Inner Panel:1 ↔ #8-32 Nylock Nut (275-1027):10
- Angle:70 (0 deg): Motor Bracket Inner Panel:1 ↔ #8-32 Nylock Nut (275-1027):9
- Angle:71 (0 deg): Motor Bracket Inner Panel:1 ↔ #8-32 Nylock Nut (275-1027):7
- Angle:72 (0 deg): Motor Bracket Inner Panel:1 ↔ #8-32 Nylock Nut (275-1027):8
- Mate:187: VersaPlanetary v2 NoStage:2 ↔ Falcon 500, Powered by Talon FX (217-6515):1
- Mate:188: VersaPlanetary v2 NoStage:5 ↔ Falcon 500, Powered by Talon FX (217-6515):5
- Mate:189: VersaPlanetary v2 NoStage Encoder:1 ↔ Falcon 500, Powered by Talon FX (217-6515):2
- Mate:190: VersaPlanetary v2 NoStage:4 ↔ Falcon 500, Powered by Talon FX (217-6515):3
- Mate:191: VersaPlanetary v2 NoStage:3 ↔ Falcon 500, Powered by Talon FX (217-6515):4
- Mate:192: VersaPlanetary v2 NoStage:3 ↔ Falcon 500, Powered by Talon FX (217-6515):4
- Mate:193: VersaPlanetary v2 NoStage:2 ↔ Falcon 500, Powered by Talon FX (217-6515):1
- Mate:194: VersaPlanetary v2 NoStage:5 ↔ Falcon 500, Powered by Talon FX (217-6515):5
- Mate:195: VersaPlanetary v2 NoStage:4 ↔ Falcon 500, Powered by Talon FX (217-6515):3
- Mate:196: VersaPlanetary v2 NoStage:3 ↔ Falcon 500, Powered by Talon FX (217-6515):4
- Mate:197: VersaPlanetary v2 NoStage:3 ↔ Falcon 500, Powered by Talon FX (217-6515):4
- Mate:198: VersaPlanetary v2 NoStage:4 ↔ Falcon 500, Powered by Talon FX (217-6515):3
- Mate:199: VersaPlanetary v2 NoStage Encoder:1 ↔ Falcon 500, Powered by Talon FX (217-6515):2
- Mate:200: VersaPlanetary v2 NoStage:2 ↔ Falcon 500, Powered by Talon FX (217-6515):1
- Mate:201: VersaPlanetary v2 NoStage:5 ↔ Falcon 500, Powered by Talon FX (217-6515):5
- Flush:12: VersaPlanetary v2 NoStage:3 ↔ VersaPlanetary v2 NoStage:4
- Mate:202: VersaPlanetary v2 NoStage:5 ↔ Motor Bracket Inner Panel:1
## Named parameters: d53_d43 = 0 mm, d54_d48 = 0 deg, d55_d23 = 0 mm, d56_d24 = 0 mm, d57_d27 = 0 mm
